# Autodesk Inventor assembly: Assembly
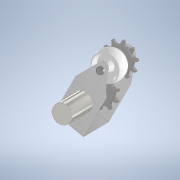
[picture p0: Inventor's stored thumbnail of the model, 180x180]
Saved by Autodesk Inventor 2020 (Build 240168000, 168)
## iProperties
Created: 2022-06-23
Part Number: Assembly
Document SubType Name: Assembly
Designer: karimi2
Author: karimi2
## Documents named in this file (6)
- C:\Users\karimi2\Documents\PROJECT\Assembly.iam
- C:\Users\karimi2\Documents\PROJECT\Frame.ipt
- C:\Users\karimi2\Documents\PROJECT\GearedDCmotor.ipt
- C:\Users\karimi2\Documents\PROJECT\casterwheel.ipt
- C:\Users\karimi2\Documents\PROJECT\wheelshaft.ipt
- C:\Users\karimi2\Documents\PROJECT\5mmSprocket.ipt
## Components (6 placed, 5 different names)
1. Frame:1 — Mate:2, Mate:3, Flush:1, Mate:7, Mate:10, Mate:12
2. GearedDCmotor:1 — Mate:3, Flush:1, Mate:4, Mate:5
3. casterwheel:1 — Mate:2, Mate:6, Mate:9, Mate:10
4. 5mmSprocket:1 — Mate:4, Mate:5
5. wheelshaft:1 — Mate:6, Mate:7, Mate:9, Mate:11
6. 5mmSprocket:2 — Mate:11, Mate:12
## Relationships (11: Mate 10, Flush 1)
- Mate:2: Frame:1 ↔ casterwheel:1
- Mate:3: Frame:1 ↔ GearedDCmotor:1
- Flush:1 (-40 mm): Frame:1 ↔ GearedDCmotor:1
- Mate:4: GearedDCmotor:1 ↔ 5mmSprocket:1
- Mate:5 (-6 mm): GearedDCmotor:1 ↔ 5mmSprocket:1
- Mate:6: casterwheel:1 ↔ wheelshaft:1
- Mate:7: Frame:1 ↔ wheelshaft:1
- Mate:9: casterwheel:1 ↔ wheelshaft:1
- Mate:10 (8 mm): Frame:1 ↔ casterwheel:1
- Mate:11: wheelshaft:1 ↔ 5mmSprocket:2
- Mate:12 (9.519 mm): Frame:1 ↔ 5mmSprocket:2
